# Autodesk Inventor assembly: Stepper-28BYJ_asm
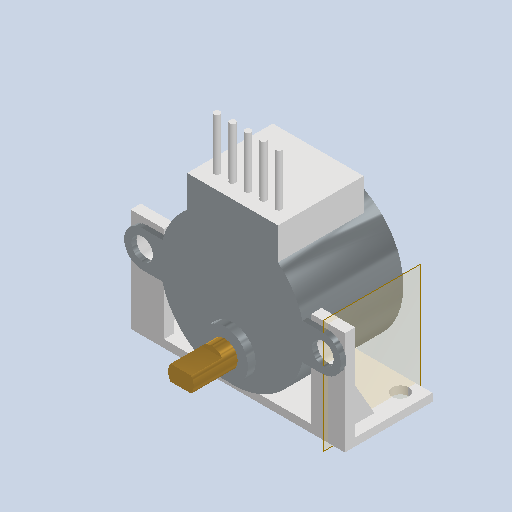
[picture p0: Inventor's stored thumbnail of the model, 512x512]
Saved by Autodesk Inventor 2025 (Build 290162000, 162)
## iProperties
Created: 2025-07-13
Part Number: Stepper-28BYJ_asm
Document SubType Name: Assembly
Designer: daisuke
Author: daisuke
## Documents named in this file (3)
- G:\マイドライブ\project\micro-mouse\3D-Model\Stepper-28BYJ_asm.iam
- G:\マイドライブ\project\micro-mouse\3D-Model\28BYJ-48_Braket.ipt
- G:\マイドライブ\project\micro-mouse\3D-Model\28BYJ-48.ipt
## Components (2 placed, 2 different names)
1. 28BYJ-48_Braket:1 — メイト:1, メイト:2, メイト:3
2. 28BYJ-48:1 — メイト:1, メイト:2, メイト:3
## Relationships (3: Mate 3)
- メイト:1 [Mate]: 28BYJ-48_Braket:1 ↔ 28BYJ-48:1
- メイト:2 [Mate]: 28BYJ-48_Braket:1 ↔ 28BYJ-48:1
- メイト:3 [Mate]: 28BYJ-48_Braket:1 ↔ 28BYJ-48:1
